# Autodesk Inventor assembly: VERSION3-small-upright-hook
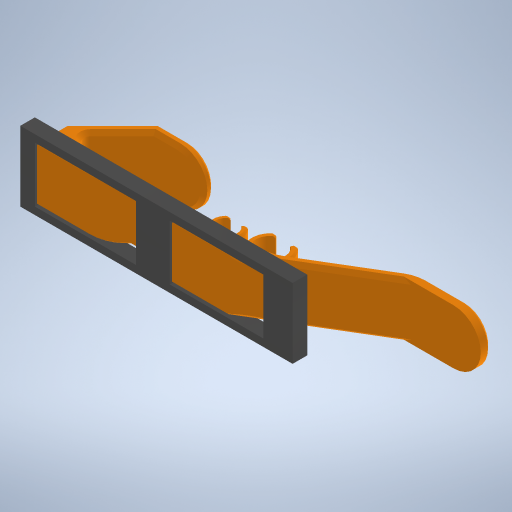
[picture p0: Inventor's stored thumbnail of the model, 512x512]
Saved by Autodesk Inventor 2024.1 (Build 281209000, 209)
## iProperties
Created: 2024-09-23
Part Number: VERSION3-small-upright-hook
Document SubType Name: Assembly
Designer: Imogen Heard
Author: Imogen Heard
## Documents named in this file (3)
- C:\Users\iwheard\Documents\0004-CAD\3D-cad-main\cable-hanger\VERSION3-small-upright-hook.iam
- C:\Users\iwheard\Documents\0004-CAD\3D-cad-main\cable-hanger\backplate-0.ipt
- C:\Users\iwheard\Documents\0004-CAD\3D-cad-main\cable-hanger\cable-hanger-dual-large.ipt
## Components (2 placed, 2 different names)
1. backplate-0:1 — Mate:2, Mate:3
2. cable-hanger-dual-large:1 — Mate:2, Mate:3
## Relationships (2: Mate 2)
- Mate:2: backplate-0:1 ↔ cable-hanger-dual-large:1
- Mate:3: backplate-0:1 ↔ cable-hanger-dual-large:1
